# Autodesk Inventor assembly: new wind guide3
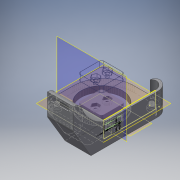
[picture p0: Inventor's stored thumbnail of the model, 180x180]
Saved by Autodesk Inventor 2016 (Build 200138000, 138)
## iProperties
Created: 2016-01-18
Part Number: new wind guide3
Document SubType Name: Assembly
Designer: Erwin Ried
Author: Erwin Ried
## Documents named in this file (3)
- D:\OneDrive\RepRap\Parts\New\new wind\HOLDER-NOT SHORT\new wind guide3.iam
- D:\OneDrive\RepRap\Parts\New\new wind\HOLDER-NOT SHORT\base.ipt
- D:\OneDrive\RepRap\Parts\New\new wind\HOLDER-NOT SHORT\little_holder.ipt
## Components (2 placed, 2 different names)
1. base:1 — Flush:1
2. little_holder:1 — Flush:1
## Relationships (1: Flush 1)
- Flush:1: base:1 ↔ little_holder:1
